# Autodesk Inventor assembly: Trebuchet
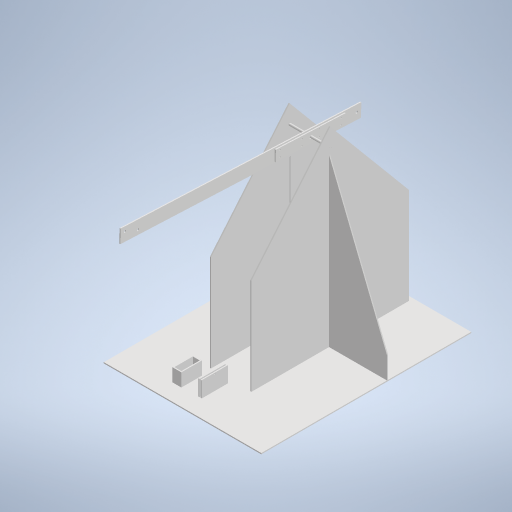
[picture p0: Inventor's stored thumbnail of the model, 512x512]
Saved by Autodesk Inventor 2023 (Build 270158000, 158)
## iProperties
Created: 2023-10-15
Part Number: Trebuchet
Document SubType Name: Assembly
Designer: Nate
Author: Nate
## Documents named in this file (10)
- C:\Users\Nate\Documents\GitHub\MMAE_232\Trebuchet\Trebuchet.iam
- C:\Users\Nate\Documents\GitHub\MMAE_232\Trebuchet\base.ipt
- C:\Users\Nate\Documents\GitHub\MMAE_232\Trebuchet\side.ipt
- C:\Users\Nate\Documents\GitHub\MMAE_232\Trebuchet\side support.ipt
- C:\Users\Nate\Documents\GitHub\MMAE_232\Trebuchet\servo long side.ipt
- C:\Users\Nate\Documents\GitHub\MMAE_232\Trebuchet\servo short side.ipt
- C:\Users\Nate\Documents\GitHub\MMAE_232\Trebuchet\pin holder.ipt
- C:\Users\Nate\Documents\GitHub\MMAE_232\Trebuchet\pin holder middle.ipt
- C:\Users\Nate\Documents\GitHub\MMAE_232\Trebuchet\arm assembly.iam
- C:\Users\Nate\Documents\GitHub\MMAE_232\Trebuchet\acrylic rod.ipt
## Components (14 placed, 9 different names)
1. base:1 — Mate:1, Mate:2, Mate:3, Mate:4, Mate:5, Mate:6, Mate:7, Mate:8, Mate:11, Mate:12, Mate:13, Mate:14, Mate:15, Mate:16, Mate:19, Mate:20, Mate:21, Mate:22, Mate:23, Mate:24, Mate:25, Mate:26
2. side:1 — Mate:3, Mate:4, Mate:27, Mate:28
3. side:2 — Mate:1, Mate:2
4. side support:1 — Mate:7, Mate:8
5. side support:2 — Mate:5, Mate:6
6. servo long side:1 — Mate:23, Mate:24
7. servo long side:2 — Mate:21, Mate:22
8. servo short side:1 — Mate:25, Mate:26
9. servo short side:2 — Mate:19, Mate:20
10. pin holder:1 — Mate:15, Mate:16
11. pin holder:2 — Mate:13, Mate:14
12. pin holder middle:1 — Mate:11, Mate:12
13. arm assembly:1 [sub-assembly] — Mate:27
14. acrylic rod:1 — Mate:28
## Relationships (24: Mate 24)
- Mate:1: base:1 ↔ side:2
- Mate:2: base:1 ↔ side:2
- Mate:3: base:1 ↔ side:1
- Mate:4: base:1 ↔ side:1
- Mate:5: base:1 ↔ side support:2
- Mate:6: base:1 ↔ side support:2
- Mate:7: base:1 ↔ side support:1
- Mate:8: base:1 ↔ side support:1
- Mate:11: base:1 ↔ pin holder middle:1
- Mate:12: base:1 ↔ pin holder middle:1
- Mate:13: base:1 ↔ pin holder:2
- Mate:14: base:1 ↔ pin holder:2
- Mate:15: base:1 ↔ pin holder:1
- Mate:16: base:1 ↔ pin holder:1
- Mate:19: base:1 ↔ servo short side:2
- Mate:20: base:1 ↔ servo short side:2
- Mate:21: base:1 ↔ servo long side:2
- Mate:22: base:1 ↔ servo long side:2
- Mate:23: base:1 ↔ servo long side:1
- Mate:24: base:1 ↔ servo long side:1
- Mate:25: base:1 ↔ servo short side:1
- Mate:26: base:1 ↔ servo short side:1
- Mate:27 (52.4129 mm): side:1 ↔ arm assembly:1
- Mate:28: side:1 ↔ acrylic rod:1
